# Autodesk Inventor assembly: LED-Spot
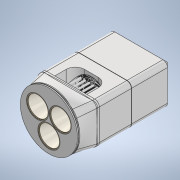
[picture p0: Inventor's stored thumbnail of the model, 180x180]
Saved by Autodesk Inventor 2021 (Build 250183000, 183)
## iProperties
Company: Open CASCADE
Created: 2026-05-21
Part Number: LED-Spot
Description: Open CASCADE Model
Document SubType Name: Assembly
Designer: Lukas
Authority: Unknown
Sending System: Open CASCADE 7.9
Preprocessor: Open CASCADE STEP processor 7.9
Title: Open CASCADE Shape Model
Author: Author
## Documents named in this file (10)
- Z:\Datastorrage\Projects\Lab-Lamp\Mechanics\LED-Spot.iam
- Z:\Datastorrage\Projects\Lab-Lamp\Mechanics\ick_s_r_28.5x18.5.ipt
- Z:\Datastorrage\Projects\Lab-Lamp\Mechanics\25x25x10_fan.ipt
- Z:\Datastorrage\Projects\Lab-Lamp\Mechanics\LED-Spot_v1.ipt
- Z:\Datastorrage\Projects\Lab-Lamp\Mechanics\Lab-Lamp_v1.ipt
- Z:\Datastorrage\Projects\Lab-Lamp\Mechanics\ICK_BGA_14_X_14_X_10.ipt
- Z:\Datastorrage\Projects\Lab-Lamp\Mechanics\Housing_Front.ipt
- Z:\Datastorrage\Projects\Lab-Lamp\Mechanics\Housing_Center.ipt
- Z:\Datastorrage\Projects\Lab-Lamp\Mechanics\Housing_Vents.ipt
- Z:\Datastorrage\Projects\Lab-Lamp\Mechanics\Housing_Top.ipt
## Components (9 placed, 9 different names)
1. LED-Spot_v1:2 — Mate:9, Angle:2, Mate:11, Mate:12, Mate:15, Flush:1, Mate:16, Angle:3, Mate:17, Mate:18, Mate:19, Mate:21, Mate:22, Mate:23, Mate:24
2. ick_s_r_28.5x18.5:1 — Mate:6, Mate:9, Angle:2, Flush:4, Mate:20
3. 25x25x10_fan:1 — Mate:6, Angle:3
4. Lab-Lamp_v1:1 — Mate:11, Mate:12, Mate:13, Mate:14, Mate:17, Mate:28, Mate:29, Mate:30
5. ICK_BGA_14_X_14_X_10:1 — Mate:13, Mate:14, Flush:2
6. Housing_Front:1 — Mate:18, Mate:19, Mate:21
7. Housing_Center:1 — Mate:22, Mate:23, Mate:24, Mate:25, Mate:26, Mate:27
8. Housing_Vents:1 — Mate:25, Mate:26, Mate:27
9. Housing_Top:1 — Mate:28, Mate:29, Mate:30
## Relationships (27: Mate 22, Flush 3, Angle 2)
- Mate:6: ick_s_r_28.5x18.5:1 ↔ 25x25x10_fan:1
- Mate:9: LED-Spot_v1:2 ↔ ick_s_r_28.5x18.5:1
- Angle:2 (0 deg): LED-Spot_v1:2 ↔ ick_s_r_28.5x18.5:1
- Mate:11: LED-Spot_v1:2 ↔ Lab-Lamp_v1:1
- Mate:12: LED-Spot_v1:2 ↔ Lab-Lamp_v1:1
- Mate:13: Lab-Lamp_v1:1 ↔ ICK_BGA_14_X_14_X_10:1
- Mate:14: Lab-Lamp_v1:1 ↔ ICK_BGA_14_X_14_X_10:1
- Mate:15: LED-Spot_v1:2
- Flush:1: LED-Spot_v1:2
- Mate:16: LED-Spot_v1:2
- Angle:3 (0 deg): LED-Spot_v1:2 ↔ 25x25x10_fan:1
- Flush:2 (7 mm): ICK_BGA_14_X_14_X_10:1
- Mate:17 (45 mm): LED-Spot_v1:2 ↔ Lab-Lamp_v1:1
- Mate:18: LED-Spot_v1:2 ↔ Housing_Front:1
- Mate:19: LED-Spot_v1:2 ↔ Housing_Front:1
- Flush:4: ick_s_r_28.5x18.5:1
- Mate:20: ick_s_r_28.5x18.5:1
- Mate:21: LED-Spot_v1:2 ↔ Housing_Front:1
- Mate:22: LED-Spot_v1:2 ↔ Housing_Center:1
- Mate:23: LED-Spot_v1:2 ↔ Housing_Center:1
- Mate:24: LED-Spot_v1:2 ↔ Housing_Center:1
- Mate:25: Housing_Center:1 ↔ Housing_Vents:1
- Mate:26: Housing_Center:1 ↔ Housing_Vents:1
- Mate:27: Housing_Center:1 ↔ Housing_Vents:1
- Mate:28: Lab-Lamp_v1:1 ↔ Housing_Top:1
- Mate:29: Lab-Lamp_v1:1 ↔ Housing_Top:1
- Mate:30: Lab-Lamp_v1:1 ↔ Housing_Top:1
